# Autodesk Inventor assembly: AssemblyNEWarm_MIR
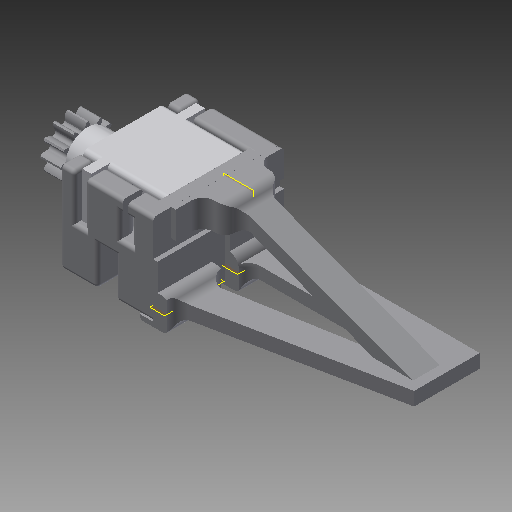
[picture p0: Inventor's stored thumbnail of the model, 512x512]
Saved by Autodesk Inventor 2018 (Build 220112000, 112)
## iProperties
Created: 2017-12-09
Part Number: AssemblyNEWarm_MIR
Document SubType Name: Assembly
Designer: reide
Author: kcmat
## Documents named in this file (7)
- C:\Users\reide\OneDrive\Documents\Inventor\TSA\2018\Animatronics\Tortoise\arms\AssemblyNEWarm_MIR.iam
- C:\Users\reide\OneDrive\Documents\Inventor\TSA\2018\Animatronics\Tortoise\arms\newShoulder_MIR.ipt
- C:\Users\reide\OneDrive\Documents\Inventor\TSA\2018\Animatronics\Tortoise\arms\straightBar_MIR.ipt
- C:\Users\reide\OneDrive\Documents\Inventor\TSA\2018\Animatronics\Tortoise\arms\AngleArm_MIR.ipt
- C:\Users\reide\OneDrive\Documents\Inventor\TSA\2018\Animatronics\Tortoise\arms\bottomARM_MIR.ipt
- C:\Users\reide\OneDrive\Documents\Inventor\TSA\2018\Animatronics\Tortoise\Mock Parts\servo (2)_MIR.ipt
- C:\Users\reide\OneDrive\Documents\Inventor\TSA\2018\Animatronics\Tortoise\Pinion final_MIR.ipt
## Components (6 placed, 6 different names)
1. newShoulder_MIR:1 — Mate:4, Mate:3, Flush:2, Mate:2, Mate:1, Flush:1, Flush:4, Flush:3, Mate:6, Flush:5, Mate:7
2. straightBar_MIR:1 — Mate:4, Mate:3, Flush:2
3. AngleArm_MIR:1 — Mate:2, Mate:1, Flush:1
4. bottomARM_MIR:1 — Flush:4, Flush:3, Mate:6
5. servo (2)_MIR:1 — Flush:5, Mate:7, Mate:9, Mate:8
6. Pinion final_MIR:1 — Mate:9, Mate:8
## Relationships (13: Mate 8, Flush 5)
- Mate:4: newShoulder_MIR:1 ↔ straightBar_MIR:1
- Mate:3: newShoulder_MIR:1 ↔ straightBar_MIR:1
- Flush:2: newShoulder_MIR:1 ↔ straightBar_MIR:1
- Mate:2: newShoulder_MIR:1 ↔ AngleArm_MIR:1
- Mate:1: newShoulder_MIR:1 ↔ AngleArm_MIR:1
- Flush:1: newShoulder_MIR:1 ↔ AngleArm_MIR:1
- Flush:4: newShoulder_MIR:1 ↔ bottomARM_MIR:1
- Flush:3: newShoulder_MIR:1 ↔ bottomARM_MIR:1
- Mate:6: newShoulder_MIR:1 ↔ bottomARM_MIR:1
- Flush:5: newShoulder_MIR:1 ↔ servo (2)_MIR:1
- Mate:7: newShoulder_MIR:1 ↔ servo (2)_MIR:1
- Mate:9: servo (2)_MIR:1 ↔ Pinion final_MIR:1
- Mate:8: servo (2)_MIR:1 ↔ Pinion final_MIR:1
